# Autodesk Inventor assembly: spielfeld_gesamt
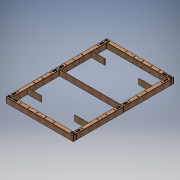
[picture p0: Inventor's stored thumbnail of the model, 180x180]
Saved by Autodesk Inventor 2016 SP2 (Build 200236200, 236)
## iProperties
Created: 2018-04-09
Part Number: spielfeld_gesamt
Document SubType Name: Assembly
Designer: wepet
Mass: 74349.4 g
Surface Area: 110381 cm^2
Volume: 74349.4 cm^3
Density: 1 g/cm^3
Author: wepet
## Documents named in this file (6)
- L:\Granz\RoboSAX\spielfeld_gesamt.iam
- L:\Granz\RoboSAX\licht_150.iam
- L:\Granz\RoboSAX\licht_200.iam
- L:\Granz\RoboSAX\licht_150_MIR.iam
- L:\Granz\RoboSAX\spielfeld_trennwand.ipt
- L:\Granz\RoboSAX\Steckwand.ipt
## Components (11 placed, 5 different names)
1. licht_150:1 [sub-assembly] — Passend:1, Fluchtend:1, Fluchtend:2, Fluchtend:3, Fluchtend:4, Einfügen:1, Einfügen:2
2. licht_150:2 [sub-assembly] — Passend:3, Fluchtend:7, Fluchtend:8, Fluchtend:9, Fluchtend:10, Fluchtend:11, Fluchtend:12, Passend:5, Einfügen:7, Einfügen:8
3. licht_200:1 [sub-assembly] — Passend:1, Fluchtend:1, Fluchtend:2, Passend:4
4. licht_200:2 [sub-assembly] — Passend:2, Fluchtend:5, Fluchtend:6, Passend:3, Fluchtend:7, Fluchtend:8
5. licht_150_MIR:1 [sub-assembly] — Fluchtend:3, Fluchtend:4, Passend:2, Fluchtend:5, Fluchtend:6, Einfügen:3, Einfügen:4
6. licht_150_MIR:2 [sub-assembly] — Fluchtend:9, Fluchtend:10, Passend:4, Passend:6, Einfügen:5, Einfügen:6
7. spielfeld_trennwand:1 — Fluchtend:11, Fluchtend:12, Passend:5, Passend:6
8. Steckwand:1 — Einfügen:1, Einfügen:2
9. Steckwand:2 — Einfügen:3, Einfügen:4
10. Steckwand:3 — Einfügen:5, Einfügen:6
11. Steckwand:4 — Einfügen:7, Einfügen:8
## Relationships (26: Flush 12, Insert 8, Mate 6)
- Passend:1 [Mate]: licht_150:1 ↔ licht_200:1
- Fluchtend:1 [Flush]: licht_150:1 ↔ licht_200:1
- Fluchtend:2 [Flush]: licht_150:1 ↔ licht_200:1
- Fluchtend:3 [Flush]: licht_150:1 ↔ licht_150_MIR:1
- Fluchtend:4 [Flush]: licht_150:1 ↔ licht_150_MIR:1
- Passend:2 [Mate]: licht_200:2 ↔ licht_150_MIR:1
- Fluchtend:5 [Flush]: licht_200:2 ↔ licht_150_MIR:1
- Fluchtend:6 [Flush]: licht_200:2 ↔ licht_150_MIR:1
- Passend:3 [Mate]: licht_150:2 ↔ licht_200:2
- Fluchtend:7 [Flush]: licht_150:2 ↔ licht_200:2
- Fluchtend:8 [Flush]: licht_150:2 ↔ licht_200:2
- Fluchtend:9 [Flush]: licht_150:2 ↔ licht_150_MIR:2
- Fluchtend:10 [Flush]: licht_150:2 ↔ licht_150_MIR:2
- Passend:4 [Mate]: licht_200:1 ↔ licht_150_MIR:2
- Fluchtend:11 [Flush]: licht_150:2 ↔ spielfeld_trennwand:1
- Fluchtend:12 [Flush]: licht_150:2 ↔ spielfeld_trennwand:1
- Passend:5 [Mate]: licht_150:2 ↔ spielfeld_trennwand:1
- Passend:6 [Mate]: licht_150_MIR:2 ↔ spielfeld_trennwand:1
- Einfügen:1 [Insert]: licht_150:1 ↔ Steckwand:1
- Einfügen:2 [Insert]: licht_150:1 ↔ Steckwand:1
- Einfügen:3 [Insert]: licht_150_MIR:1 ↔ Steckwand:2
- Einfügen:4 [Insert]: licht_150_MIR:1 ↔ Steckwand:2
- Einfügen:5 [Insert]: licht_150_MIR:2 ↔ Steckwand:3
- Einfügen:6 [Insert]: licht_150_MIR:2 ↔ Steckwand:3
- Einfügen:7 [Insert]: licht_150:2 ↔ Steckwand:4
- Einfügen:8 [Insert]: licht_150:2 ↔ Steckwand:4
